# Autodesk Inventor assembly: Mould assembly
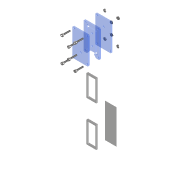
[picture p0: Inventor's stored thumbnail of the model, 180x180]
Saved by Autodesk Inventor 2020 (Build 240168000, 168)
## iProperties
Created: 2022-03-07
Part Number: Mould assembly
Document SubType Name: Assembly
Designer: ferrerx
Author: ferrerx
## Documents named in this file (8)
- C:\Users\ferrerx\Documents\GitHub\Embryo-micro-injection-vessel\Design files\Mould assembly.iam
- C:\Users\ferrerx\Documents\GitHub\Embryo-micro-injection-vessel\Design files\Middle external.ipt
- C:\Users\ferrerx\Documents\GitHub\Embryo-micro-injection-vessel\Design files\Middle internal.ipt
- C:\Users\ferrerx\Documents\GitHub\Embryo-micro-injection-vessel\Design files\Top&Bottom.ipt
- C:\Users\ferrerx\Documents\Inventor\Content Center Files\R2020\en-US\ANSI B18.3.1M(1)\ANSI B18.3.1M - M3x0.5 x 16(2).ipt
- C:\Users\ferrerx\Documents\Inventor\Content Center Files\R2020\en-US\AS 1474(1)\AS 1474 - M3(1).ipt
- C:\Users\ferrerx\Documents\GitHub\Embryo-micro-injection-vessel\Design files\Chamber.ipt
- C:\Users\ferrerx\Documents\GitHub\Embryo-micro-injection-vessel\Design files\Coverslip.ipt
## Components (19 placed, 7 different names)
1. Middle external:1 — Mate:3, Mate:4, Flush:1, Mate:19, Flush:2
2. Middle internal:1 — Mate:1, Mate:2, Flush:1
3. Top&Bottom:1 — Mate:5, Mate:6, Mate:7, Mate:8, Mate:9, Mate:10, Mate:11, Mate:12
4. Top&Bottom:2 — Mate:1, Mate:2, Mate:3, Mate:4, Mate:5, Mate:6, Mate:13, Mate:14, Mate:15, Mate:16, Mate:17, Mate:18
5. Broached Socket Head Cap Screw - Metric M3x0.5 x 16:1 — Mate:7
6. Broached Socket Head Cap Screw - Metric M3x0.5 x 16:2 — Mate:9
7. Broached Socket Head Cap Screw - Metric M3x0.5 x 16:3 — Mate:11
8. Broached Socket Head Cap Screw - Metric M3x0.5 x 16:4 — Mate:12
9. Broached Socket Head Cap Screw - Metric M3x0.5 x 16:5 — Mate:8
10. Broached Socket Head Cap Screw - Metric M3x0.5 x 16:6 — Mate:10
11. AS 1474 - Metric M3:1 — Mate:13
12. AS 1474 - Metric M3:2 — Mate:14
13. AS 1474 - Metric M3:3 — Mate:15
14. AS 1474 - Metric M3:4 — Mate:16
15. AS 1474 - Metric M3:5 — Mate:17
16. AS 1474 - Metric M3:6 — Mate:18
17. Chamber:1 — Mate:19, Flush:2, Flush:3, Flush:4
18. Chamber:2 — Flush:3, Flush:4, Flush:5
19. Coverslip:1 — Flush:5
## Relationships (24: Mate 19, Flush 5)
- Mate:1: Middle internal:1 ↔ Top&Bottom:2
- Mate:2: Middle internal:1 ↔ Top&Bottom:2
- Mate:3: Middle external:1 ↔ Top&Bottom:2
- Mate:4: Middle external:1 ↔ Top&Bottom:2
- Mate:5: Top&Bottom:1 ↔ Top&Bottom:2
- Mate:6: Top&Bottom:1 ↔ Top&Bottom:2
- Flush:1: Middle external:1 ↔ Middle internal:1
- Mate:7: Top&Bottom:1 ↔ Broached Socket Head Cap Screw - Metric M3x0.5 x 16:1
- Mate:8: Top&Bottom:1 ↔ Broached Socket Head Cap Screw - Metric M3x0.5 x 16:5
- Mate:9: Top&Bottom:1 ↔ Broached Socket Head Cap Screw - Metric M3x0.5 x 16:2
- Mate:10: Top&Bottom:1 ↔ Broached Socket Head Cap Screw - Metric M3x0.5 x 16:6
- Mate:11: Top&Bottom:1 ↔ Broached Socket Head Cap Screw - Metric M3x0.5 x 16:3
- Mate:12: Top&Bottom:1 ↔ Broached Socket Head Cap Screw - Metric M3x0.5 x 16:4
- Mate:13: Top&Bottom:2 ↔ AS 1474 - Metric M3:1
- Mate:14: Top&Bottom:2 ↔ AS 1474 - Metric M3:2
- Mate:15: Top&Bottom:2 ↔ AS 1474 - Metric M3:3
- Mate:16: Top&Bottom:2 ↔ AS 1474 - Metric M3:4
- Mate:17: Top&Bottom:2 ↔ AS 1474 - Metric M3:5
- Mate:18: Top&Bottom:2 ↔ AS 1474 - Metric M3:6
- Mate:19: Middle external:1 ↔ Chamber:1
- Flush:2: Middle external:1 ↔ Chamber:1
- Flush:3: Chamber:1 ↔ Chamber:2
- Flush:4: Chamber:1 ↔ Chamber:2
- Flush:5 (1 mm): Chamber:2 ↔ Coverslip:1
